# Autodesk Inventor assembly: exp1
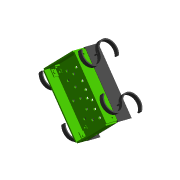
[picture p0: Inventor's stored thumbnail of the model, 180x180]
Saved by Autodesk Inventor 2019 (Build 230136000, 136)
## iProperties
Part Number: exp1
Document SubType Name: Assembly
Designer: Ranjita
Author: Ranjita
## Documents named in this file (6)
- D:\mechanical tutorial\exp1.iam
- C:\Users\Ranjita\Documents\Inventor\Content Center Files\R2019\base2.ipt
- C:\Users\Ranjita\Documents\Inventor\Content Center Files\R2019\mooootoooor.ipt
- C:\Users\Ranjita\Documents\Inventor\Content Center Files\R2019\transparent base.ipt
- C:\Users\Ranjita\Documents\Inventor\Content Center Files\R2019\leg of model.iam
- C:\Users\Ranjita\Documents\Inventor\Content Center Files\R2019\leg of model2.iam
## Components (10 placed, 5 different names)
1. base2:1 — Rotational:1, Rotational:2, Rotational:3, Rotational:4, Rigid:1
2. mooootoooor:1 — Rotational:1, Rotational:5
3. mooootoooor:2 — Rotational:2, Rotational:7
4. mooootoooor:3 — Rotational:4, Rotational:8
5. mooootoooor:4 — Rotational:3, Rotational:6
6. transparent base:1 — Rigid:1
7. leg of model:1 [sub-assembly] — Rotational:6
8. leg of model:2 [sub-assembly] — Rotational:5
9. leg of model2:1 [sub-assembly] — Rotational:8
10. leg of model2:2 [sub-assembly] — Rotational:7
## Relationships (9: RevoluteJoint 8, WeldJoint 1)
- Rotational:1 [RevoluteJoint]: base2:1 ↔ mooootoooor:1
- Rotational:2 [RevoluteJoint]: base2:1 ↔ mooootoooor:2
- Rotational:3 [RevoluteJoint]: base2:1 ↔ mooootoooor:4
- Rotational:4 [RevoluteJoint]: base2:1 ↔ mooootoooor:3
- Rigid:1 [WeldJoint]: base2:1 ↔ transparent base:1
- Rotational:5 [RevoluteJoint]: mooootoooor:1 ↔ leg of model:2
- Rotational:6 [RevoluteJoint]: mooootoooor:4 ↔ leg of model:1
- Rotational:7 [RevoluteJoint]: mooootoooor:2 ↔ leg of model2:2
- Rotational:8 [RevoluteJoint]: mooootoooor:3 ↔ leg of model2:1
